# Autodesk Inventor assembly: Wheel Orientation
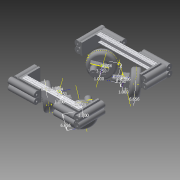
[picture p0: Inventor's stored thumbnail of the model, 180x180]
Saved by Autodesk Inventor 2015 (Build 190159000, 159)
## iProperties
Created: 2016-01-19
Part Number: Wheel Orientation
Document SubType Name: Assembly
Designer: sethbattis
Author: sethbattis
## Documents named in this file (6)
- \\area51\team3566\cad\FRC 2016\Space Claims.iam
- \\area51\team3566\cad\FRC 2016\Wheelbase.ipt
- \\area51\team3566\cad\FRC 2016\Snow Tire Wheel with Gearbox and CIM.ipt
- \\area51\team3566\cad\FRC 2016\Basic Frame.ipt
- \\area51\team3566\cad\FRC 2016\Corner Bumper.ipt
- \\area51\team3566\cad\FRC 2016\AM14U3 End Sheet 24.5in.ipt
## Components (12 placed, 5 different names)
1. Wheelbase:1 — Rotational:1, Rotational:2, Rotational:3, Rotational:4, Flush:1, Rigid:1
2. Snow Tire Wheel with Gearbox and CIM:1 — Rotational:2
3. Snow Tire Wheel with Gearbox and CIM:2 — Rotational:1
4. Snow Tire Wheel with Gearbox and CIM:3 — Rotational:4
5. Snow Tire Wheel with Gearbox and CIM:4 — Rotational:3
6. Basic Frame:1 — Flush:1, Rigid:1, Mate:1, Mate:2, Flush:2, Flush:3, Flush:4, Flush:5, Mate:3, Mate:4, Flush:6, Flush:7, Flush:8, Flush:9, Mate:5, Flush:10, Flush:11, Mate:10, Mate:11, Flush:12
7. Corner Bumper:1 — Mate:1, Mate:3, Flush:6
8. Corner Bumper:2 — Mate:2, Flush:2, Flush:7
9. Corner Bumper:3 — Flush:4, Mate:4, Flush:9
10. Corner Bumper:4 — Flush:3, Flush:5, Flush:8
11. AM14U3 End Sheet 24.5in:1 — Flush:10, Flush:11, Mate:10
12. AM14U3 End Sheet 24.5in:2 — Mate:5, Mate:11, Flush:12
## Relationships (24: Flush 12, Mate 7, RevoluteJoint 4, WeldJoint 1)
- Rotational:1 [RevoluteJoint]: Wheelbase:1 ↔ Snow Tire Wheel with Gearbox and CIM:2
- Rotational:2 [RevoluteJoint]: Wheelbase:1 ↔ Snow Tire Wheel with Gearbox and CIM:1
- Rotational:3 [RevoluteJoint]: Wheelbase:1 ↔ Snow Tire Wheel with Gearbox and CIM:4
- Rotational:4 [RevoluteJoint]: Wheelbase:1 ↔ Snow Tire Wheel with Gearbox and CIM:3
- Flush:1: Wheelbase:1 ↔ Basic Frame:1
- Rigid:1 [WeldJoint]: Wheelbase:1 ↔ Basic Frame:1
- Mate:1: Basic Frame:1 ↔ Corner Bumper:1
- Mate:2: Basic Frame:1 ↔ Corner Bumper:2
- Flush:2: Basic Frame:1 ↔ Corner Bumper:2
- Flush:3: Basic Frame:1 ↔ Corner Bumper:4
- Flush:4: Basic Frame:1 ↔ Corner Bumper:3
- Flush:5: Basic Frame:1 ↔ Corner Bumper:4
- Mate:3: Basic Frame:1 ↔ Corner Bumper:1
- Mate:4: Basic Frame:1 ↔ Corner Bumper:3
- Flush:6: Basic Frame:1 ↔ Corner Bumper:1
- Flush:7: Basic Frame:1 ↔ Corner Bumper:2
- Flush:8: Basic Frame:1 ↔ Corner Bumper:4
- Flush:9: Basic Frame:1 ↔ Corner Bumper:3
- Mate:5: Basic Frame:1 ↔ AM14U3 End Sheet 24.5in:2
- Flush:10: Basic Frame:1 ↔ AM14U3 End Sheet 24.5in:1
- Flush:11: Basic Frame:1 ↔ AM14U3 End Sheet 24.5in:1
- Mate:10: Basic Frame:1 ↔ AM14U3 End Sheet 24.5in:1
- Mate:11: Basic Frame:1 ↔ AM14U3 End Sheet 24.5in:2
- Flush:12: Basic Frame:1 ↔ AM14U3 End Sheet 24.5in:2
